# Autodesk Inventor assembly: Sujetador Porta Suero
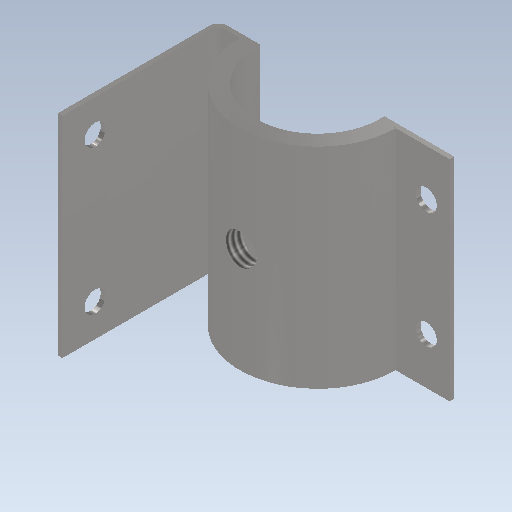
[picture p0: Inventor's stored thumbnail of the model, 512x512]
Saved by Autodesk Inventor 2020.3 (Build 243373000, 373)
## iProperties
Created: 2020-06-30
Part Number: Sujetador Porta Suero
Document SubType Name: Assembly
Designer: Bruno
Author: Bruno
## Documents named in this file (4)
- C:\Users\Bruno\Desktop\CNAF\CNAF-3\Sujetador Porta Suero.iam
- C:\Users\Bruno\Desktop\CNAF\CNAF-3\Sujeta Porta Suero-sin tubo.ipt
- C:\Users\Bruno\Desktop\CNAF\CNAF-3\Half Pipe A53 - DN25-H45.ipt
- C:\Users\Bruno\Desktop\CNAF\CNAF-3\Pletina Terminal V2.ipt
## Components (3 placed, 3 different names)
1. Sujeta Porta Suero-sin tubo:1 — Mate:1, Flush:1, Tangent:1
2. Half Pipe A53 - DN25-H45:1 — Mate:1, Flush:1, Tangent:1, Flush:2
3. Pletina Terminal V2:1 — Flush:2
## Relationships (4: Flush 2, Mate 1, Tangent 1)
- Mate:1: Sujeta Porta Suero-sin tubo:1 ↔ Half Pipe A53 - DN25-H45:1
- Flush:1: Sujeta Porta Suero-sin tubo:1 ↔ Half Pipe A53 - DN25-H45:1
- Tangent:1: Sujeta Porta Suero-sin tubo:1 ↔ Half Pipe A53 - DN25-H45:1
- Flush:2: Half Pipe A53 - DN25-H45:1 ↔ Pletina Terminal V2:1
